# Autodesk Inventor assembly: HarmonicDriveProto1
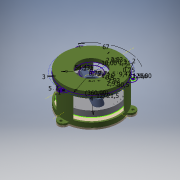
[picture p0: Inventor's stored thumbnail of the model, 180x180]
Saved by Autodesk Inventor 2018.3 (Build 223284000, 284)
## iProperties
Created: 2018-07-02
Part Number: HarmonicDriveProto1
Material: Generisch
Document SubType Name: Assembly
Designer: JochenAlt
Author: JochenAlt
## Documents named in this file (3)
- D:\Projects\FlowerPot\CAD\HarmonicDriveProto1.iam
- D:\Projects\FlowerPot\CAD\HarmonicDriveProto1.ipt
- D:\Projects\FlowerPot\CAD\HarmonicDriveWaveGenerator-Proto1.ipt
## Components (2 placed, 2 different names)
1. Harmonic Drive:1 — Passend:1
2. HarmonicDriveWaveGenerator-Proto1:1 — Passend:1
## Relationships (1: Mate 1)
- Passend:1 [Mate]: Harmonic Drive:1 ↔ HarmonicDriveWaveGenerator-Proto1:1
